# Autodesk Inventor assembly: hinge_assembly
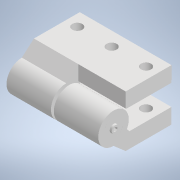
[picture p0: Inventor's stored thumbnail of the model, 180x180]
Saved by Autodesk Inventor 2021 (Build 250183000, 183)
## iProperties
Created: 2023-12-08
Part Number: hinge_assembly
Document SubType Name: Assembly
Designer: assman
Author: assman
## Documents named in this file (3)
- D:\3DPrinting\3DModels\roco\hinge_assembly.iam
- D:\3DPrinting\3DModels\roco\hinge_01.ipt
- D:\3DPrinting\3DModels\roco\hinge_02.ipt
## Components (2 placed, 2 different names)
1. hinge_01:1 — Rotational:1
2. hinge_02:1 — Rotational:1
## Relationships (1: RevoluteJoint 1)
- Rotational:1 [RevoluteJoint]: hinge_01:1 ↔ hinge_02:1
